# Autodesk Inventor assembly: Assembly1
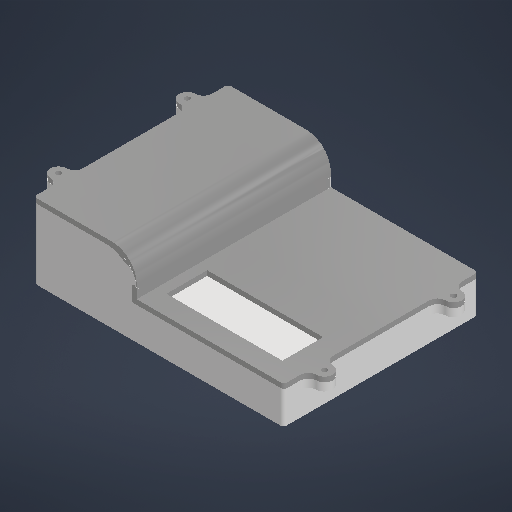
[picture p0: Inventor's stored thumbnail of the model, 512x512]
Saved by Autodesk Inventor 2026.1 (Build 301233020, 233B)
## iProperties
Created: 2026-07-01
Part Number: Assembly1
Document SubType Name: Assembly
Designer: Asus
Author: Asus
## Documents named in this file (3)
- D:\1_projects\KKN\landfill-air-quality-monitoring-system-\aquos_chasis\Assembly1.iam
- D:\1_projects\KKN\landfill-air-quality-monitoring-system-\aquos_chasis\base.ipt
- D:\1_projects\KKN\landfill-air-quality-monitoring-system-\aquos_chasis\top.ipt
## Components (2 placed, 2 different names)
1. base:1 — Rigid:1, Rigid:2
2. top:1 — Rigid:1, Rigid:2
## Relationships (2: WeldJoint 2)
- Rigid:1 [WeldJoint]: base:1 ↔ top:1
- Rigid:2 [WeldJoint]: base:1 ↔ top:1
